# Autodesk Inventor assembly: nc_omuni_1
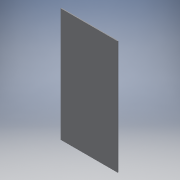
[picture p0: Inventor's stored thumbnail of the model, 180x180]
Saved by Autodesk Inventor 2019 (Build 230136000, 136)
## iProperties
Created: 2022-03-17
Part Number: nc_omuni_1
Material: 一般
Document SubType Name: Assembly
Designer: yuta
Author: yuta
## Documents named in this file (4)
- C:\Users\yuta\Documents\NHK\nc_omuni_1.iam
- C:\Users\yuta\Documents\NHK\NC.port.ipt
- C:\Users\yuta\Downloads\オムニホイール\オムニホイール\ホイールユニット_モータ固定板.ipt
- C:\Users\yuta\Downloads\オムニホイール\オムニホイール\ホイールユニット_エンコーダ取付板.ipt
## Components (3 placed, 3 different names)
1. NC.port:1 — メイト:1, フラッシュ:1, フラッシュ:2, メイト:2, フラッシュ:3
2. ホイールユニット_モータ固定板:1 — メイト:1, フラッシュ:1, フラッシュ:2, メイト:3
3. ホイールユニット_エンコーダ取付板:1 — メイト:2, フラッシュ:3, メイト:3
## Relationships (6: Mate 3, Flush 3)
- メイト:1 [Mate]: NC.port:1 ↔ ホイールユニット_モータ固定板:1
- フラッシュ:1 [Flush] (6 mm): NC.port:1 ↔ ホイールユニット_モータ固定板:1
- フラッシュ:2 [Flush] (6 mm): NC.port:1 ↔ ホイールユニット_モータ固定板:1
- メイト:2 [Mate]: NC.port:1 ↔ ホイールユニット_エンコーダ取付板:1
- フラッシュ:3 [Flush] (6 mm): NC.port:1 ↔ ホイールユニット_エンコーダ取付板:1
- メイト:3 [Mate] (22 mm): ホイールユニット_モータ固定板:1 ↔ ホイールユニット_エンコーダ取付板:1
